# Autodesk Inventor assembly: Flywheel
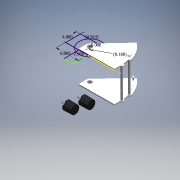
[picture p0: Inventor's stored thumbnail of the model, 180x180]
Saved by Autodesk Inventor 2018 (Build 220112000, 112)
## iProperties
Created: 2020-01-19
Part Number: Flywheel
Document SubType Name: Assembly
Designer: Victor
Author: Victor
## Documents named in this file (6)
- E:\Downloads\GrabCAD\Infinite Recharge 2020\Build season\Flywheel\Flywheel.iam
- E:\Downloads\GrabCAD\Infinite Recharge 2020\Build season\Flywheel\Hood rod.ipt
- E:\Downloads\GrabCAD\Deep Space 2019\Build Season\Chassis\217-2731_0_500_flanged_bearing.ipt
- E:\Downloads\GrabCAD\Infinite Recharge 2020\Build season\Flywheel\Hood panel RIGHT .ipt
- E:\Downloads\GrabCAD\Infinite Recharge 2020\Build season\Flywheel\Hood panel LEFT.ipt
- E:\Downloads\GrabCAD\Deep Space 2019\Build Season\CLB_Rear_Motor.iam
## Components (8 placed, 5 different names)
1. Hood rod:1 — Insert:4, Insert:7
2. Hood rod:4 — Insert:2, Insert:8
3. 217-2731_0_500_flanged_bearing:1 — Insert:9
4. 217-2731_0_500_flanged_bearing:2 — Insert:6
5. Hood panel RIGHT :1 — Insert:2, Insert:4, Insert:6
6. Hood panel LEFT:1 — Insert:7, Insert:8, Insert:9
7. CLB_Rear_Motor:1 [sub-assembly]
8. CLB_Rear_Motor:2 [sub-assembly]
## Relationships (6: Insert 6)
- Insert:2: Hood rod:4 ↔ Hood panel RIGHT :1
- Insert:4: Hood rod:1 ↔ Hood panel RIGHT :1
- Insert:6: 217-2731_0_500_flanged_bearing:2 ↔ Hood panel RIGHT :1
- Insert:7: Hood rod:1 ↔ Hood panel LEFT:1
- Insert:8: Hood rod:4 ↔ Hood panel LEFT:1
- Insert:9: 217-2731_0_500_flanged_bearing:1 ↔ Hood panel LEFT:1
